# Autodesk Inventor assembly: gear
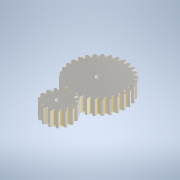
[picture p0: Inventor's stored thumbnail of the model, 180x180]
Saved by Autodesk Inventor 2021 (Build 250183000, 183)
## iProperties
Created: 2021-04-12
Part Number: gear
Document SubType Name: Assembly
Designer: Jawal
Author: Jawal
## Documents named in this file (3)
- C:\Users\Jawal\Documents\UNI\PART III\Semester 1\MECHENG 334\Project A\CAD Files\Main\Main_Assembly_export\gear.iam
- C:\Users\Jawal\Documents\UNI\PART III\Semester 1\MECHENG 334\Project A\CAD Files\Main\Main_Assembly_export\Spur Gear12.ipt
- C:\Users\Jawal\Documents\UNI\PART III\Semester 1\MECHENG 334\Project A\CAD Files\Main\Main_Assembly_export\Final Spur Gear Large.ipt
## Components (2 placed, 2 different names)
1. Spur Gear1:1 — Mate:2, Flush:2, Tangent:1, Rotation:1
2. Spur Gear2:1 — Flush:1, Mate:1, Tangent:1, Rotation:1
## Relationships (6: Flush 2, Mate 2, Tangent 1, RelateRotation 1)
- Flush:1: Spur Gear2:1
- Mate:1: Spur Gear2:1
- Mate:2: Spur Gear1:1
- Flush:2: Spur Gear1:1
- Tangent:1: Spur Gear1:1 ↔ Spur Gear2:1
- Rotation:1 [RelateRotation] (2 ul): Spur Gear1:1 ↔ Spur Gear2:1
